# Autodesk Inventor assembly: power-splitter-plate
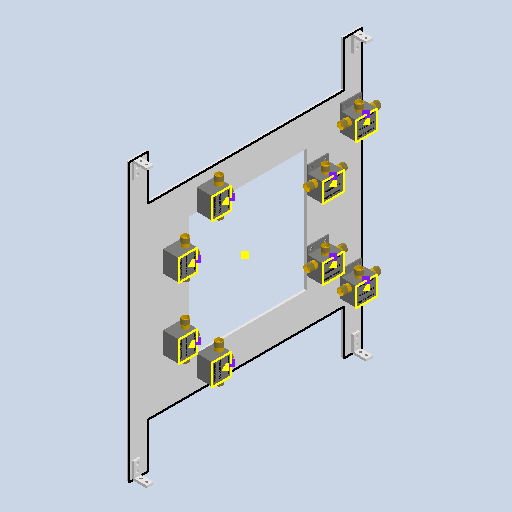
[picture p0: Inventor's stored thumbnail of the model, 512x512]
Saved by Autodesk Inventor 2024 (Build 280153000, 153)
## iProperties
Created: 2023-10-02
Part Number: power-splitter-plate
Document SubType Name: Assembly
Designer: Alexander Pollak
Author: Alexander Pollak
## Documents named in this file (4)
- C:\Users\Alexander Pollak\ownCloud\Inventor\ATA_2019\ATA_IF_PowerSplitter_6U\Custom Parts\power-splitter-plate.iam
- C:\Users\Alexander Pollak\ownCloud\Inventor\ATA_2019\ATA_IF_PowerSplitter_6U\Custom Parts\24567474_200.ipt
- C:\Users\Alexander Pollak\ownCloud\Inventor\ATA_2019\Shared_Parts\ZX10-2-12-S+\ZX10-2-12-S+.iam
- C:\Users\Alexander Pollak\ownCloud\Inventor\ATA_2019\ATA_IF_PowerSplitter_6U\Custom Parts\24567474_201.ipt
## Components (13 placed, 3 different names)
1. 24567474_200:1 — Insert:1, Insert:2, Insert:3, Insert:4, Insert:5, Insert:6, Insert:7, Insert:8, Insert:9, Insert:10, Insert:11, Insert:12, Insert:13, Insert:14, Insert:15, Insert:16, Insert:17, Insert:18, Insert:19, Insert:20, Insert:21, Insert:22, Insert:23, Insert:24
2. ZX10-2-12-S+:8 [sub-assembly] — Insert:9, Insert:10
3. ZX10-2-12-S+:7 [sub-assembly] — Insert:11, Insert:12
4. ZX10-2-12-S+:6 [sub-assembly] — Insert:13, Insert:14
5. ZX10-2-12-S+:5 [sub-assembly] — Insert:15, Insert:16
6. ZX10-2-12-S+:4 [sub-assembly] — Insert:1, Insert:2
7. ZX10-2-12-S+:3 [sub-assembly] — Insert:3, Insert:4
8. ZX10-2-12-S+:2 [sub-assembly] — Insert:5, Insert:6
9. ZX10-2-12-S+:1 [sub-assembly] — Insert:7, Insert:8
10. 24567474_201:1 — Insert:23, Insert:24
11. 24567474_201:2 — Insert:21, Insert:22
12. 24567474_201:3 — Insert:19, Insert:20
13. 24567474_201:4 — Insert:17, Insert:18
## Relationships (24: Insert 24)
- Insert:1: 24567474_200:1 ↔ ZX10-2-12-S+:4
- Insert:2: 24567474_200:1 ↔ ZX10-2-12-S+:4
- Insert:3: 24567474_200:1 ↔ ZX10-2-12-S+:3
- Insert:4: 24567474_200:1 ↔ ZX10-2-12-S+:3
- Insert:5: 24567474_200:1 ↔ ZX10-2-12-S+:2
- Insert:6: 24567474_200:1 ↔ ZX10-2-12-S+:2
- Insert:7: 24567474_200:1 ↔ ZX10-2-12-S+:1
- Insert:8: 24567474_200:1 ↔ ZX10-2-12-S+:1
- Insert:9: 24567474_200:1 ↔ ZX10-2-12-S+:8
- Insert:10: 24567474_200:1 ↔ ZX10-2-12-S+:8
- Insert:11: 24567474_200:1 ↔ ZX10-2-12-S+:7
- Insert:12: 24567474_200:1 ↔ ZX10-2-12-S+:7
- Insert:13: 24567474_200:1 ↔ ZX10-2-12-S+:6
- Insert:14: 24567474_200:1 ↔ ZX10-2-12-S+:6
- Insert:15: 24567474_200:1 ↔ ZX10-2-12-S+:5
- Insert:16: 24567474_200:1 ↔ ZX10-2-12-S+:5
- Insert:17: 24567474_200:1 ↔ 24567474_201:4
- Insert:18: 24567474_200:1 ↔ 24567474_201:4
- Insert:19: 24567474_200:1 ↔ 24567474_201:3
- Insert:20: 24567474_200:1 ↔ 24567474_201:3
- Insert:21: 24567474_200:1 ↔ 24567474_201:2
- Insert:22: 24567474_200:1 ↔ 24567474_201:2
- Insert:23: 24567474_200:1 ↔ 24567474_201:1
- Insert:24: 24567474_200:1 ↔ 24567474_201:1
